# Autodesk Inventor assembly: Secondary Regulator Assembly
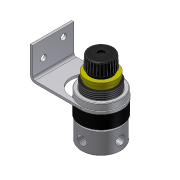
[picture p0: Inventor's stored thumbnail of the model, 180x180]
Saved by Autodesk Inventor 2013 (Build 170138000, 138)
## iProperties
Category: Pneumatics
Shininess: 64.0
Length Units: 11269
Angle Units: 11279
Time Units: 11290
Mass Units: 11283
Length Display Precision: 3
Angle Display Precision: 2
Compacted: True
Created: 2005-01-09
Document SubType Name: Assembly
Manufacturer: Standard
Standards Organization: Custom
Description: Secondary Regulator Assembly
Vendor: Monnier
Project: FIRST
Density: 0.0
Volumn: 0.0
Area: 0.0
PropertySet Name: Model Information
Control State: 0
Master: False
Checked Out: False
Title: Secondary Regulator Assembly
Author: Autodesk, Inc.
## Documents named in this file (4)
- C:\Users\Moses\Documents\GitHub\frc2013CAD\Pneumatics\Pneumatics_Monnier_101-3002-1_Assembly.iam
- C:\Users\Moses\Documents\GitHub\frc2013CAD\Pneumatics\Pneumatics_Monnier_101-3002-1.ipt
- C:\Users\Moses\Documents\GitHub\frc2013CAD\Pneumatics\Pneumatics_Monnier_13536_Mounting Bracket.ipt
- C:\Users\Moses\Documents\GitHub\frc2013CAD\Pneumatics\Pneumatics_Monnier_13536_Mounting Ring.ipt
## Components (3 placed, 3 different names)
1. Pneumatics_Monnier_101-3002-1:1 — Mate:1, Mate:2, Transitional:1
2. Pneumatics_Monnier_13536_Mounting Bracket:1 — Mate:2, Transitional:1, Mate:3
3. Pneumatics_Monnier_13536_Mounting Ring:1 — Mate:1, Mate:3
## Relationships (4: Mate 3, Transitional 1)
- Mate:1: Pneumatics_Monnier_101-3002-1:1 ↔ Pneumatics_Monnier_13536_Mounting Ring:1
- Mate:2: Pneumatics_Monnier_101-3002-1:1 ↔ Pneumatics_Monnier_13536_Mounting Bracket:1
- Transitional:1: Pneumatics_Monnier_101-3002-1:1 ↔ Pneumatics_Monnier_13536_Mounting Bracket:1
- Mate:3: Pneumatics_Monnier_13536_Mounting Bracket:1 ↔ Pneumatics_Monnier_13536_Mounting Ring:1
